# Autodesk Inventor assembly: Drive V3
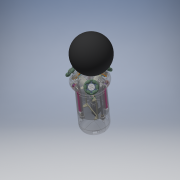
[picture p0: Inventor's stored thumbnail of the model, 180x180]
Saved by Autodesk Inventor 2019.1 (Build 231200000, 200)
## iProperties
Created: 2018-06-30
Part Number: Drive V3
Material: Generisch
Document SubType Name: Assembly
Designer: JochenAlt
Author: JochenAlt
## Documents named in this file (6)
- D:\Projects\Ondine\CAD\Drive V4.iam
- D:\Projects\Ondine\CAD\Sphere.ipt
- D:\Projects\Ondine\CAD\DriveChain V4.iam
- D:\Projects\Ondine\CAD\PCB\ControllerPCBHolder.ipt
- D:\Projects\Ondine\CAD\SpindleMotor.iam
- D:\Projects\Ondine\CAD\LegMotorHolder.ipt
## Components (7 placed, 5 different names)
1. Sphere:1 — Passend:38, Tangential:1
2. DriveChain V4:1 [sub-assembly] — Passend:53, Passend:56
3. DriveChain V4:2 [sub-assembly] — Passend:54, Passend:55, Passend:56, Tangential:1, Passend:57
4. DriveChain V4:3 [sub-assembly] — Passend:53, Passend:54, Passend:55, Passend:58, Passend:59, Passend:60, Passend:61, Fluchtend:1
5. PCBHolder:1 — Passend:57, Passend:58
6. SpindleMotor:1 [sub-assembly] — Passend:52, Fluchtend:1
7. LegMotorHolder:1 — Passend:52, Passend:59, Passend:60, Passend:61
## Relationships (13: Mate 11, Tangent 1, Flush 1)
- Passend:38 [Mate]: Sphere:1
- Passend:52 [Mate]: SpindleMotor:1 ↔ LegMotorHolder:1
- Passend:53 [Mate]: DriveChain V4:1 ↔ DriveChain V4:3
- Passend:54 [Mate]: DriveChain V4:2 ↔ DriveChain V4:3
- Passend:55 [Mate]: DriveChain V4:2 ↔ DriveChain V4:3
- Passend:56 [Mate]: DriveChain V4:1 ↔ DriveChain V4:2
- Tangential:1: Sphere:1 ↔ DriveChain V4:2
- Passend:57 [Mate]: DriveChain V4:2 ↔ PCBHolder:1
- Passend:58 [Mate]: DriveChain V4:3 ↔ PCBHolder:1
- Passend:59 [Mate]: DriveChain V4:3 ↔ LegMotorHolder:1
- Passend:60 [Mate]: DriveChain V4:3 ↔ LegMotorHolder:1
- Passend:61 [Mate]: DriveChain V4:3 ↔ LegMotorHolder:1
- Fluchtend:1 [Flush]: DriveChain V4:3 ↔ SpindleMotor:1
